# Autodesk Inventor assembly: Front bar with Motors_MIR
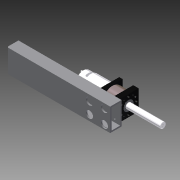
[picture p0: Inventor's stored thumbnail of the model, 180x180]
Saved by Autodesk Inventor 2015 (Build 190159000, 159)
## iProperties
Created: 2015-01-21
Part Number: Front bar with Motors_MIR
Document SubType Name: Assembly
Designer: chapale16
Author: chapale16
## Documents named in this file (3)
- \\lhssvr02\Homedirs\Robotics Club\CAD Model 2015\Front bar with Motors_MIR.iam
- \\lhssvr02\Homedirs\Robotics Club\CAD Model 2015\Modified Front Frame 27 in_MIR.ipt
- \\lhssvr02\Homedirs\Robotics Club\CAD Model 2015\Parts Folder\Gear Boxes\Bane Bots\16-1\BB-42016.iam
## Components (2 placed, 2 different names)
1. Modified Front Frame 27 in_MIR:1 — Angle:1, Insert:1
2. BB-42016:1 [sub-assembly] — Angle:1, Insert:1
## Relationships (2: Angle 1, Insert 1)
- Angle:1 (0 deg): Modified Front Frame 27 in_MIR:1 ↔ BB-42016:1
- Insert:1: Modified Front Frame 27 in_MIR:1 ↔ BB-42016:1
